# Autodesk Inventor assembly: Ensamble
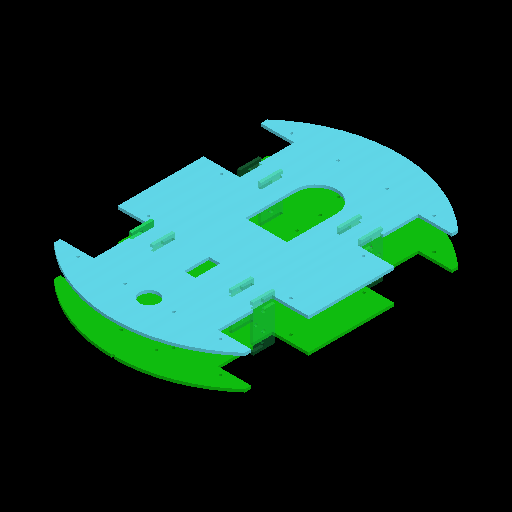
[picture p0: Inventor's stored thumbnail of the model, 512x512]
Saved by Autodesk Inventor 2025.2 (Build 292293000, 293)
## iProperties
Created: 2024-12-02
Part Number: Ensamble
Document SubType Name: Assembly
Designer: braughton
Author: braughton
## Documents named in this file (4)
- I:\2025-1\DM\ProyectoFinal\Omnidirectional-self-driven-car\Ensamble.iam
- I:\2025-1\DM\ProyectoFinal\Omnidirectional-self-driven-car\ChasisInferior.ipt
- I:\2025-1\DM\ProyectoFinal\Omnidirectional-self-driven-car\ChasisSuperior.ipt
- I:\2025-1\DM\ProyectoFinal\Omnidirectional-self-driven-car\SoporteMotor.ipt
## Components (10 placed, 3 different names)
1. ChasisInferior:1 — Flush:1, Mate:1, Mate:2, Flush:4, Flush:5, Flush:6, Mate:3, Mate:4, Mate:5, Mate:6, Mate:7, Mate:8, Flush:10, Flush:7, Flush:11, Flush:12, Mate:9, Mate:10, Mate:11, Mate:12, Mate:13, Mate:14, Mate:15, Mate:16
2. ChasisSuperior:1 — Flush:13, Mate:17, Mate:18
3. SoporteMotor:1 — Flush:1, Mate:1, Mate:2, Mate:17, Mate:18
4. SoporteMotor:2 — Flush:5, Mate:5, Mate:6
5. SoporteMotor:3 — Flush:6, Mate:7, Mate:8
6. SoporteMotor:4 — Flush:4, Mate:3, Mate:4
7. SoporteMotor:5 — Flush:10, Mate:13, Mate:14
8. SoporteMotor:6 — Flush:11, Mate:11, Mate:12
9. SoporteMotor:7 — Flush:12, Mate:9, Mate:10, Flush:13
10. SoporteMotor:8 — Flush:7, Mate:15, Mate:16
## Relationships (27: Mate 18, Flush 9)
- Flush:1: ChasisInferior:1 ↔ SoporteMotor:1
- Mate:1: ChasisInferior:1 ↔ SoporteMotor:1
- Mate:2: ChasisInferior:1 ↔ SoporteMotor:1
- Flush:4: ChasisInferior:1 ↔ SoporteMotor:4
- Flush:5: ChasisInferior:1 ↔ SoporteMotor:2
- Flush:6: ChasisInferior:1 ↔ SoporteMotor:3
- Mate:3: ChasisInferior:1 ↔ SoporteMotor:4
- Mate:4: ChasisInferior:1 ↔ SoporteMotor:4
- Mate:5: ChasisInferior:1 ↔ SoporteMotor:2
- Mate:6: ChasisInferior:1 ↔ SoporteMotor:2
- Mate:7: ChasisInferior:1 ↔ SoporteMotor:3
- Mate:8: ChasisInferior:1 ↔ SoporteMotor:3
- Flush:10: ChasisInferior:1 ↔ SoporteMotor:5
- Flush:7: ChasisInferior:1 ↔ SoporteMotor:8
- Flush:11: ChasisInferior:1 ↔ SoporteMotor:6
- Flush:12: ChasisInferior:1 ↔ SoporteMotor:7
- Mate:9: ChasisInferior:1 ↔ SoporteMotor:7
- Mate:10: ChasisInferior:1 ↔ SoporteMotor:7
- Mate:11: ChasisInferior:1 ↔ SoporteMotor:6
- Mate:12: ChasisInferior:1 ↔ SoporteMotor:6
- Mate:13: ChasisInferior:1 ↔ SoporteMotor:5
- Mate:14: ChasisInferior:1 ↔ SoporteMotor:5
- Mate:15: ChasisInferior:1 ↔ SoporteMotor:8
- Mate:16: ChasisInferior:1 ↔ SoporteMotor:8
- Flush:13: ChasisSuperior:1 ↔ SoporteMotor:7
- Mate:17: ChasisSuperior:1 ↔ SoporteMotor:1
- Mate:18: ChasisSuperior:1 ↔ SoporteMotor:1
